# Autodesk Inventor assembly: Link_00_Assembly_V02
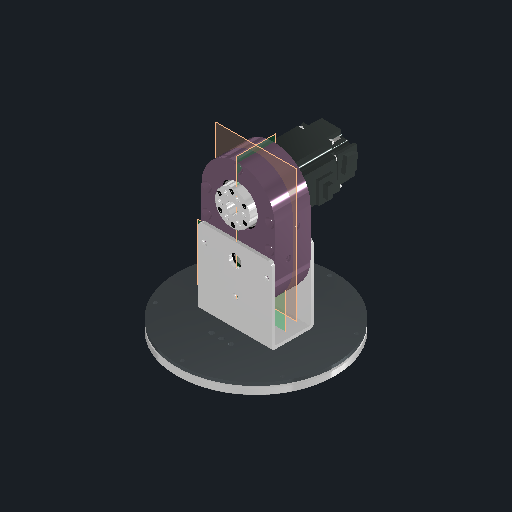
[picture p0: Inventor's stored thumbnail of the model, 512x512]
Saved by Autodesk Inventor 2026 (Build 300175000, 175)
## iProperties
Created: 2025-12-01
Part Number: Link_00_Assembly_V02
Document SubType Name: Assembly
Designer: DanielFGarzon
Mass: 1941.18 g
Surface Area: 3803.65 cm^2
Volume: 1082.81 cm^3
Author: DanielFGarzon
## Documents named in this file (9)
- D:\POLIMI\3RD SEMESTER\Industrial Robotics\Project\Mine\Link_00_Assembly_V02.iam
- D:\POLIMI\3RD SEMESTER\Industrial Robotics\Project\Mine\Shaft_02.ipt
- D:\POLIMI\3RD SEMESTER\Industrial Robotics\Project\Mine\FlangeHub.ipt
- D:\POLIMI\3RD SEMESTER\Industrial Robotics\Project\Mine\3M120T.ipt
- D:\POLIMI\3RD SEMESTER\Industrial Robotics\Project\Mine\Plate.ipt
- D:\POLIMI\3RD SEMESTER\Industrial Robotics\Project\Mine\Spacer_05.ipt
- D:\POLIMI\3RD SEMESTER\Industrial Robotics\Project\Mine\TurnableBearing.ipt
- D:\POLIMI\3RD SEMESTER\Industrial Robotics\Project\Mine\Fold.ipt
- D:\POLIMI\3RD SEMESTER\Industrial Robotics\Project\Mine\Reducer.iam
## Components (13 placed, 8 different names)
1. Shaft_02:1 — Mate:1, Mate:2, Flush:1, Mate:3, Mate:4
2. FlangeHub:1 — Flush:1, Mate:3, Mate:5, Mate:6, Mate:7, Mate:8
3. 3M120T:1 — Mate:4, Mate:5
4. Plate:1 — Mate:6, Mate:7, Mate:8, Mate:9, Mate:10, Mate:11, Mate:12, Mate:13, Mate:14, Mate:15, Mate:16, Mate:17, Mate:18, Mate:19, Mate:20, Mate:24, Mate:30, Mate:31
5. Spacer_05:1 — Mate:12, Mate:20, Mate:22
6. Spacer_05:2 — Mate:11, Mate:18
7. Spacer_05:3 — Mate:14, Mate:17
8. Spacer_05:4 — Mate:9, Mate:19, Mate:23
9. Spacer_05:5 — Mate:10, Mate:16, Mate:21
10. Spacer_05:6 — Mate:13, Mate:15
11. TurnableBearing:1 — Mate:21, Mate:22, Mate:23
12. Fold:1 — Mate:24, Flush:2, Mate:27, Mate:28, Mate:29, Mate:30, Mate:31
13. Reducer:1 [sub-assembly] — Mate:27, Mate:28, Mate:29
## Relationships (32: Mate 29, Flush 3)
- Mate:1: Shaft_02:1
- Mate:2: Shaft_02:1
- Flush:1: Shaft_02:1 ↔ FlangeHub:1
- Mate:3: Shaft_02:1 ↔ FlangeHub:1
- Mate:4: Shaft_02:1 ↔ 3M120T:1
- Mate:5 (2 mm): FlangeHub:1 ↔ 3M120T:1
- Mate:6: FlangeHub:1 ↔ Plate:1
- Mate:7: FlangeHub:1 ↔ Plate:1
- Mate:8: FlangeHub:1 ↔ Plate:1
- Mate:9: Plate:1 ↔ Spacer_05:4
- Mate:10: Plate:1 ↔ Spacer_05:5
- Mate:11: Plate:1 ↔ Spacer_05:2
- Mate:12: Plate:1 ↔ Spacer_05:1
- Mate:13: Plate:1 ↔ Spacer_05:6
- Mate:14: Plate:1 ↔ Spacer_05:3
- Mate:15: Plate:1 ↔ Spacer_05:6
- Mate:16: Plate:1 ↔ Spacer_05:5
- Mate:17: Plate:1 ↔ Spacer_05:3
- Mate:18: Plate:1 ↔ Spacer_05:2
- Mate:19: Plate:1 ↔ Spacer_05:4
- Mate:20: Plate:1 ↔ Spacer_05:1
- Mate:21: Spacer_05:5 ↔ TurnableBearing:1
- Mate:22: Spacer_05:1 ↔ TurnableBearing:1
- Mate:23: Spacer_05:4 ↔ TurnableBearing:1
- Mate:24: Plate:1 ↔ Fold:1
- Flush:2 (-26.8 mm): Fold:1
- Mate:27: Fold:1 ↔ Reducer:1
- Mate:28: Fold:1 ↔ Reducer:1
- Mate:29: Fold:1 ↔ Reducer:1
- Flush:3
- Mate:30: Plate:1 ↔ Fold:1
- Mate:31: Plate:1 ↔ Fold:1
